# Autodesk Inventor assembly: MotorMount_New
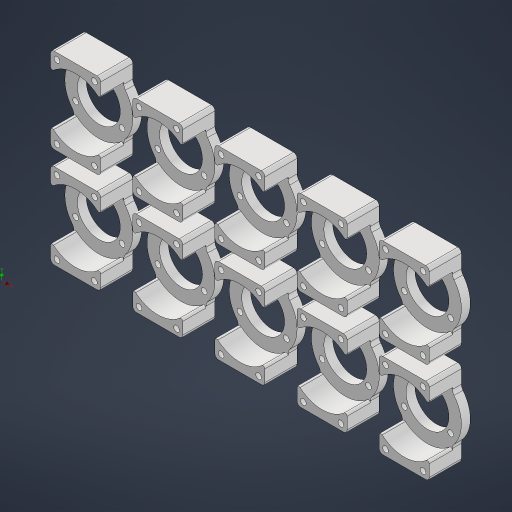
[picture p0: Inventor's stored thumbnail of the model, 512x512]
Saved by Autodesk Inventor 2024.2 (Build 282272000, 272)
## iProperties
Created: 2024-03-01
Part Number: MotorMount_New
Document SubType Name: Assembly
Designer: Hanaoka
Author: Hanaoka
## Documents named in this file (2)
- G:\共有ドライブ\reRo\05_個人\hanaoka\inventor\CAMpath\MotorMount_New.iam
- G:\共有ドライブ\reRo\05_個人\hanaoka\inventor\DriveUnit\MotorMount_sub.ipt
## Components (10 placed, 1 different names)
1. MotorMount_sub:1 — メイト:1, メイト:2, 正接:1
2. MotorMount_sub:2
3. MotorMount_sub:3
4. MotorMount_sub:4
5. MotorMount_sub:5
6. MotorMount_sub:6
7. MotorMount_sub:7
8. MotorMount_sub:8
9. MotorMount_sub:9
10. MotorMount_sub:10
## Component patterns: (10 elements, first: MotorMount_sub:1)
## Relationships (3: Mate 2, Tangent 1)
- メイト:1 [Mate]: MotorMount_sub:1
- メイト:2 [Mate]: MotorMount_sub:1
- 正接:1 [Tangent]: MotorMount_sub:1
